# Autodesk Inventor assembly: TA-ASM-1002
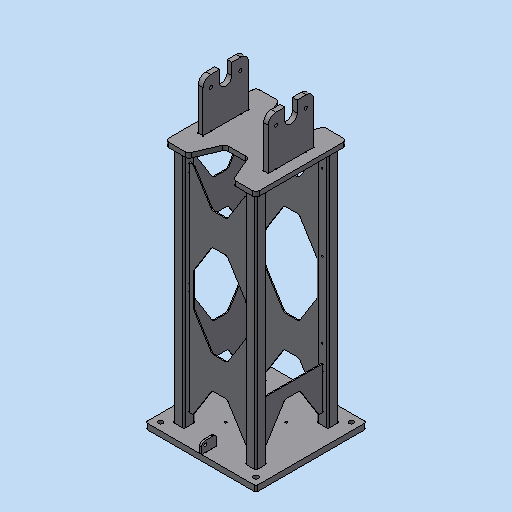
[picture p0: Inventor's stored thumbnail of the model, 512x512]
Saved by Autodesk Inventor 2025.3 (Build 293356030, 356C)
## iProperties
RuleStatus: InUse
Created: 2025-09-18
Part Number: TA-ASM-1002
Document SubType Name: Assembly
Designer: titus
Description: Weldment, Cleaning Robot Tower
Mass: 50696.9 g
Surface Area: 20397.6 cm^2
Volume: 6458.2 cm^3
Density: 7.85 g/cm^3
Author: titus
## Documents named in this file (11)
- R:\A1- Neuweg Design Data\OM Robotics\CLEANING ROBOT TOWER PROJECT\TA-ASM-1002.iam
- R:\A1- Neuweg Design Data\OM Robotics\CLEANING ROBOT TOWER PROJECT\Tower Base.ipt
- R:\A1- Neuweg Design Data\OM Robotics\CLEANING ROBOT TOWER PROJECT\Tower Top Plate.ipt
- R:\A1- Neuweg Design Data\OM Robotics\CLEANING ROBOT TOWER PROJECT\Arm Mount Plate.ipt
- R:\A1- Neuweg Design Data\OM Robotics\CLEANING ROBOT TOWER PROJECT\Tower Actuator Mount Tab.ipt
- R:\A1- Neuweg Design Data\OM Robotics\CLEANING ROBOT TOWER PROJECT\Corner Post.ipt
- R:\A1- Neuweg Design Data\OM Robotics\CLEANING ROBOT TOWER PROJECT\Tower Cross Support.ipt
- R:\A1- Neuweg Design Data\OM Robotics\CLEANING ROBOT TOWER PROJECT\Corner Post 2.ipt
- R:\A1- Neuweg Design Data\OM Robotics\CLEANING ROBOT TOWER PROJECT\Corner Post 3.ipt
- R:\A1- Neuweg Design Data\OM Robotics\CLEANING ROBOT TOWER PROJECT\Corner Post 4.ipt
- R:\A1- Neuweg Design Data\OM Robotics\CLEANING ROBOT TOWER PROJECT\Half cross support.ipt
## Components (13 placed, 10 different names)
1. Tower Base
2. Tower Top Plate:1
3. Arm Mount Plate:1
4. Tower Actuator Mount Tab:1
5. Corner Post:1
6. Arm Mount Plate:2
7. Corner Post 2:1
8. Corner Post 3:1
9. Corner Post 4:1
10. Half cross support:1
11. Tower Cross Support:1
12. Tower Cross Support:2
13. Tower Cross Support:3
## Component patterns: (3 elements, first: Tower Cross Support:1)
## Relationships (3: Flush 2, Mate 1)
- [Mate]: Tower Top Plate:1 ↔ Arm Mount Plate:2
- [Flush]: Arm Mount Plate:1 ↔ Arm Mount Plate:2
- [Flush] (34.925 mm): Tower Top Plate:1 ↔ Arm Mount Plate:2
## Named parameters: d3_d2 = 0 mm
